# Autodesk Inventor assembly: ForkLift
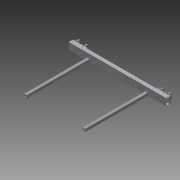
[picture p0: Inventor's stored thumbnail of the model, 180x180]
Saved by Autodesk Inventor 2015 (Build 190159000, 159)
## iProperties
Created: 2015-01-25
Part Number: ForkLift
Document SubType Name: Assembly
Designer: cstewart1
Author: cstewart1
## Documents named in this file (4)
- C:\Users\jhirshland1\Inventor\HWRobot2015CAD\Elevator\ForkLift.iam
- C:\Users\jhirshland1\Inventor\HWRobot2015CAD\Elevator\ElevatorCar.iam
- C:\Users\jhirshland1\Inventor\HWRobot2015CAD\StaticForks.ipt
- C:\Users\jhirshland1\Inventor\HWRobot2015CAD\fake.ipt
## Components (4 placed, 3 different names)
1. ElevatorCar:1 [sub-assembly] — Flush:1, Mate:1, Flush:2, Flush:3, Mate:3
2. StaticForks:1 — Flush:1, Mate:1, Mate:2, Mate:4
3. fake:1 — Flush:2, Mate:2
4. StaticForks:2 — Flush:3, Mate:3, Mate:4
## Relationships (7: Mate 4, Flush 3)
- Flush:1: ElevatorCar:1 ↔ StaticForks:1
- Mate:1: ElevatorCar:1 ↔ StaticForks:1
- Flush:2: ElevatorCar:1 ↔ fake:1
- Mate:2 (132.5626 mm): StaticForks:1 ↔ fake:1
- Flush:3: ElevatorCar:1 ↔ StaticForks:2
- Mate:3: ElevatorCar:1 ↔ StaticForks:2
- Mate:4 (406.4 mm): StaticForks:1 ↔ StaticForks:2
